# Autodesk Inventor assembly: Unidade_de_potencia
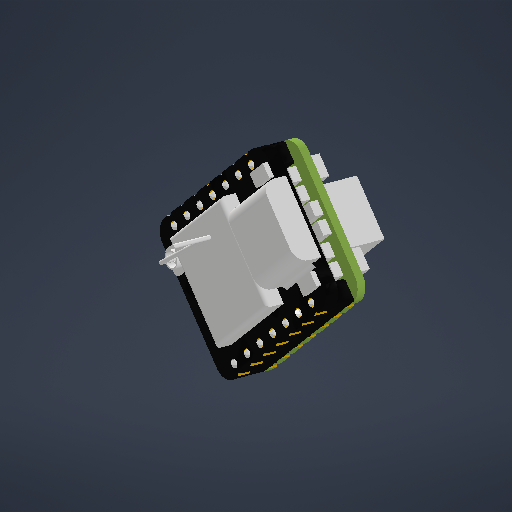
[picture p0: Inventor's stored thumbnail of the model, 512x512]
Saved by Autodesk Inventor 2027 (Build 310192000, 192)
## iProperties
Created: 2026-07-17
Part Number: Unidade_de_potencia
Document SubType Name: Assembly
Designer: marcu
Mass: 2.10691 g
Surface Area: 29.6224 cm^2
Volume: 2.10691 cm^3
Density: 1 g/cm^3
Author: marcu
## Documents named in this file (5)
- C:\Users\marcu\projetos\cin-maker\Projeto_drone\Placas_Eletrônicas.iam
- Placas_Eletrônicas.iam
- C:\Users\marcu\projetos\cin-maker\Projeto_drone\ESP32-S3.ipt
- C:\Users\marcu\projetos\cin-maker\Projeto_drone\Barra de pinos.ipt
- C:\Users\marcu\projetos\cin-maker\Projeto_drone\PCB.ipt
## Components (4 placed, 3 different names)
1. ESP32-S3:1 — Coincidente:1, Coincidente:2, Coincidente:3, Coincidente:4, Coincidente:5, Coincidente:6, Coincidente:7, Coincidente:8, Coincidente:9, Coincidente:10, Coincidente:11, Coincidente:12, Coincidente:13, Coincidente:14, Coincidente:15, Coincidente:16, Coincidente:17, Coincidente:18, Coincidente:19, Coincidente:20, Coincidente:21, Coincidente:22, Coincidente:23, Coincidente:24, Coincidente:25, Coincidente:26, Coincidente:27, Coincidente:28, Coincidente:29, Coincidente:30
2. Barra de pinos:1 — Coincidente:1, Coincidente:2, Coincidente:3, Coincidente:4, Coincidente:5, Coincidente:6, Coincidente:7, Coincidente:8, Coincidente:24, Coincidente:25, Coincidente:26, Coincidente:27, Coincidente:28, Coincidente:29, Coincidente:30, Coincidente:31, Coincidente:45, Coincidente:46, Coincidente:47, Coincidente:48, Coincidente:49, Coincidente:50, Coincidente:51, Coincidente:52, Coincidente:53, Coincidente:54, Coincidente:55, Coincidente:56, Coincidente:57, Coincidente:58
3. Barra de pinos:2 — Coincidente:9, Coincidente:10, Coincidente:11, Coincidente:12, Coincidente:13, Coincidente:14, Coincidente:15, Coincidente:16, Coincidente:17, Coincidente:18, Coincidente:19, Coincidente:20, Coincidente:21, Coincidente:22, Coincidente:23, Coincidente:32, Coincidente:33, Coincidente:34, Coincidente:35, Coincidente:36, Coincidente:37, Coincidente:38, Coincidente:39, Coincidente:40, Coincidente:41, Coincidente:42, Coincidente:43, Coincidente:44
4. PCB:1 — Coincidente:31, Coincidente:32, Coincidente:33, Coincidente:34, Coincidente:35, Coincidente:36, Coincidente:37, Coincidente:38, Coincidente:39, Coincidente:40, Coincidente:41, Coincidente:42, Coincidente:43, Coincidente:44, Coincidente:45, Coincidente:46, Coincidente:47, Coincidente:48, Coincidente:49, Coincidente:50, Coincidente:51, Coincidente:52, Coincidente:53, Coincidente:54, Coincidente:55, Coincidente:56, Coincidente:57, Coincidente:58
## Relationships (58: Mate 58)
- Coincidente:1 [Mate]: ESP32-S3:1 ↔ Barra de pinos:1
- Coincidente:2 [Mate] (-0.32 mm): ESP32-S3:1 ↔ Barra de pinos:1
- Coincidente:3 [Mate] (-0.32 mm): ESP32-S3:1 ↔ Barra de pinos:1
- Coincidente:4 [Mate] (-0.32 mm): ESP32-S3:1 ↔ Barra de pinos:1
- Coincidente:5 [Mate] (-0.32 mm): ESP32-S3:1 ↔ Barra de pinos:1
- Coincidente:6 [Mate] (-0.32 mm): ESP32-S3:1 ↔ Barra de pinos:1
- Coincidente:7 [Mate] (-0.32 mm): ESP32-S3:1 ↔ Barra de pinos:1
- Coincidente:8 [Mate] (-0.32 mm): ESP32-S3:1 ↔ Barra de pinos:1
- Coincidente:9 [Mate]: ESP32-S3:1 ↔ Barra de pinos:2
- Coincidente:10 [Mate] (-0.32 mm): ESP32-S3:1 ↔ Barra de pinos:2
- Coincidente:11 [Mate] (-0.32 mm): ESP32-S3:1 ↔ Barra de pinos:2
- Coincidente:12 [Mate] (-0.32 mm): ESP32-S3:1 ↔ Barra de pinos:2
- Coincidente:13 [Mate] (-0.32 mm): ESP32-S3:1 ↔ Barra de pinos:2
- Coincidente:14 [Mate] (-0.32 mm): ESP32-S3:1 ↔ Barra de pinos:2
- Coincidente:15 [Mate] (-0.32 mm): ESP32-S3:1 ↔ Barra de pinos:2
- Coincidente:16 [Mate] (-0.32 mm): ESP32-S3:1 ↔ Barra de pinos:2
- Coincidente:17 [Mate] (-0.32 mm): ESP32-S3:1 ↔ Barra de pinos:2
- Coincidente:18 [Mate] (-0.32 mm): ESP32-S3:1 ↔ Barra de pinos:2
- Coincidente:19 [Mate] (-0.32 mm): ESP32-S3:1 ↔ Barra de pinos:2
- Coincidente:20 [Mate] (-0.32 mm): ESP32-S3:1 ↔ Barra de pinos:2
- Coincidente:21 [Mate] (-0.32 mm): ESP32-S3:1 ↔ Barra de pinos:2
- Coincidente:22 [Mate] (-0.32 mm): ESP32-S3:1 ↔ Barra de pinos:2
- Coincidente:23 [Mate] (-0.32 mm): ESP32-S3:1 ↔ Barra de pinos:2
- Coincidente:24 [Mate] (-0.32 mm): ESP32-S3:1 ↔ Barra de pinos:1
- Coincidente:25 [Mate] (-0.32 mm): ESP32-S3:1 ↔ Barra de pinos:1
- Coincidente:26 [Mate] (-0.32 mm): ESP32-S3:1 ↔ Barra de pinos:1
- Coincidente:27 [Mate] (-0.32 mm): ESP32-S3:1 ↔ Barra de pinos:1
- Coincidente:28 [Mate] (-0.32 mm): ESP32-S3:1 ↔ Barra de pinos:1
- Coincidente:29 [Mate] (-0.32 mm): ESP32-S3:1 ↔ Barra de pinos:1
- Coincidente:30 [Mate] (-0.32 mm): ESP32-S3:1 ↔ Barra de pinos:1
- Coincidente:31 [Mate]: Barra de pinos:1 ↔ PCB:1
- Coincidente:32 [Mate] (-0.32 mm): Barra de pinos:2 ↔ PCB:1
- Coincidente:33 [Mate] (-0.32 mm): Barra de pinos:2 ↔ PCB:1
- Coincidente:34 [Mate] (-0.32 mm): Barra de pinos:2 ↔ PCB:1
- Coincidente:35 [Mate] (-0.32 mm): Barra de pinos:2 ↔ PCB:1
- Coincidente:36 [Mate] (-0.32 mm): Barra de pinos:2 ↔ PCB:1
- Coincidente:37 [Mate] (-0.32 mm): Barra de pinos:2 ↔ PCB:1
- Coincidente:38 [Mate] (-0.32 mm): Barra de pinos:2 ↔ PCB:1
- Coincidente:39 [Mate] (-0.32 mm): Barra de pinos:2 ↔ PCB:1
- Coincidente:40 [Mate] (-0.32 mm): Barra de pinos:2 ↔ PCB:1
- Coincidente:41 [Mate] (-0.32 mm): Barra de pinos:2 ↔ PCB:1
- Coincidente:42 [Mate] (-0.32 mm): Barra de pinos:2 ↔ PCB:1
- Coincidente:43 [Mate] (-0.32 mm): Barra de pinos:2 ↔ PCB:1
- Coincidente:44 [Mate] (-0.32 mm): Barra de pinos:2 ↔ PCB:1
- Coincidente:45 [Mate] (-0.32 mm): Barra de pinos:1 ↔ PCB:1
- Coincidente:46 [Mate] (-0.32 mm): Barra de pinos:1 ↔ PCB:1
- Coincidente:47 [Mate] (-0.32 mm): Barra de pinos:1 ↔ PCB:1
- Coincidente:48 [Mate] (-0.32 mm): Barra de pinos:1 ↔ PCB:1
- Coincidente:49 [Mate] (-0.32 mm): Barra de pinos:1 ↔ PCB:1
- Coincidente:50 [Mate] (-0.32 mm): Barra de pinos:1 ↔ PCB:1
- Coincidente:51 [Mate] (-0.32 mm): Barra de pinos:1 ↔ PCB:1
- Coincidente:52 [Mate] (-0.32 mm): Barra de pinos:1 ↔ PCB:1
- Coincidente:53 [Mate] (-0.32 mm): Barra de pinos:1 ↔ PCB:1
- Coincidente:54 [Mate] (-0.32 mm): Barra de pinos:1 ↔ PCB:1
- Coincidente:55 [Mate] (-0.32 mm): Barra de pinos:1 ↔ PCB:1
- Coincidente:56 [Mate] (-0.32 mm): Barra de pinos:1 ↔ PCB:1
- Coincidente:57 [Mate] (-0.32 mm): Barra de pinos:1 ↔ PCB:1
- Coincidente:58 [Mate] (-0.32 mm): Barra de pinos:1 ↔ PCB:1
## Named parameters: Finish10_Area = 0.151335, Finish10_Thickness = 0.008 mm, Finish11_Area = 0.281252, Finish11_Thickness = 0.008 mm, Finish12_Area = 0.00485813, Finish12_Thickness = 0.008 mm, Finish13_Area = 2.5981, Finish13_Thickness = 0.008 mm, Finish14_Area = 2.31685, Finish14_Thickness = 0.008 mm, Finish1_Area = 1.55962, Finish1_Thickness = 0.008 mm, Finish2_Area = 3.58025, Finish2_Thickness = 0.008 mm, Finish3_Area = 0.900008, Finish3_Thickness = 0.008 mm, Finish4_Area = 3.78041, Finish4_Thickness = 0.008 mm, Finish5_Area = 0.03841, Finish5_Thickness = 0.008 mm, Finish6_Area = 1.05097, Finish6_Thickness = 0.008 mm, Finish7_Area = 2.99464, Finish7_Thickness = 0.008 mm, Finish8_Area = 2.41913, Finish8_Thickness = 0.008 mm, Finish9_Area = 0.178491, Finish9_Thickness = 0.008 mm
note: some values were not read from the file. Shown as the stored number, unit unknown: "Finish10_Area", "Finish11_Area", "Finish12_Area", "Finish13_Area", "Finish14_Area", "Finish1_Area", "Finish2_Area", "Finish3_Area", "Finish4_Area", "Finish5_Area", "Finish6_Area", "Finish7_Area", "Finish8_Area", "Finish9_Area".
